# Autodesk Inventor assembly: GuideDemo
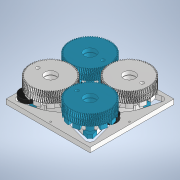
[picture p0: Inventor's stored thumbnail of the model, 180x180]
Saved by Autodesk Inventor 2020.2 (Build 242310000, 310)
## iProperties
Created: 2020-09-20
Part Number: GuideDemo
Document SubType Name: Assembly
Designer: elmar
Author: elmar
## Documents named in this file (6)
- D:\FourWireBraidingMachine\Documentation\GuideDemo.iam
- D:\FourWireBraidingMachine\InventorFiles\GuidePlateV1.ipt
- D:\FourWireBraidingMachine\InventorFiles\TipSpring.ipt
- D:\FourWireBraidingMachine\InventorFiles\HornGear.ipt
- D:\FourWireBraidingMachine\InventorFiles\HornGearMirror.ipt
- D:\FourWireBraidingMachine\InventorFiles\CarriagePlate.ipt
## Components (13 placed, 5 different names)
1. GuidePlateV1:1 — Flush:1, Mate:1, Insert:1, Insert:2, Insert:3, Insert:4, Mate:2, Mate:3, Mate:4, Mate:5, Mate:6, Mate:7, Mate:8
2. HornGear:1 — Insert:3, Angle:2, Angle:3
3. HornGear:2 — Insert:4, Angle:2
4. HornGearMirror:1 — Insert:1, Angle:1, Angle:3
5. HornGearMirror:2 — Insert:2, Angle:1
6. CarriagePlate:1 — Mate:2
7. CarriagePlate:2 — Mate:3, Mate:4
8. CarriagePlate:3
9. CarriagePlate:4 — Mate:5
10. TipSpring:1 — Flush:1, Mate:1
11. TipSpring:2
12. TipSpring:3
13. TipSpring:4
## Component patterns: (4 elements, first: TipSpring:1)
## Relationships (16: Mate 8, Insert 4, Angle 3, Flush 1)
- Flush:1: GuidePlateV1:1 ↔ TipSpring:1
- Mate:1: GuidePlateV1:1 ↔ TipSpring:1
- Insert:1 (11 mm): GuidePlateV1:1 ↔ HornGearMirror:1
- Insert:2 (11 mm): GuidePlateV1:1 ↔ HornGearMirror:2
- Insert:3 (11 mm): GuidePlateV1:1 ↔ HornGear:1
- Insert:4 (11 mm): GuidePlateV1:1 ↔ HornGear:2
- Angle:1 (180 deg): HornGearMirror:1 ↔ HornGearMirror:2
- Angle:2 (180 deg): HornGear:1 ↔ HornGear:2
- Mate:2: GuidePlateV1:1 ↔ CarriagePlate:1
- Mate:3: GuidePlateV1:1 ↔ CarriagePlate:2
- Mate:4: GuidePlateV1:1 ↔ CarriagePlate:2
- Mate:5: GuidePlateV1:1 ↔ CarriagePlate:4
- Angle:3 (0 deg): HornGear:1 ↔ HornGearMirror:1
- Mate:6: GuidePlateV1:1
- Mate:7: GuidePlateV1:1
- Mate:8: GuidePlateV1:1
